# Autodesk Inventor assembly: ModuleFold
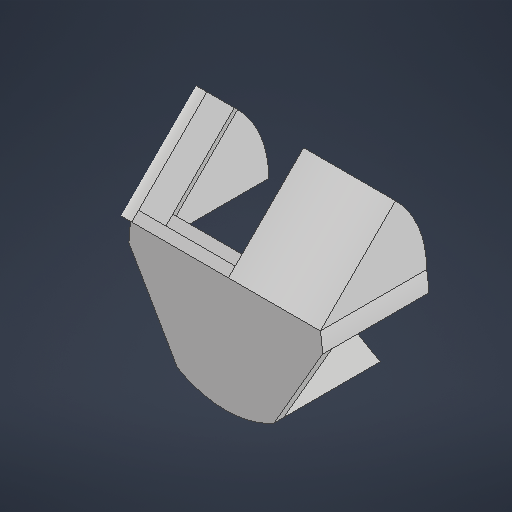
[picture p0: Inventor's stored thumbnail of the model, 512x512]
Saved by Autodesk Inventor 2026.2 (Build 302298000, 298)
## iProperties
Created: 2026-06-17
Part Number: ModuleFold
Document SubType Name: Assembly
Designer: Jakub Schmidt
Author: Jakub Schmidt
## Documents named in this file (3)
- C:\Users\Jakub Schmidt\Desktop\100M_SA\SG\10mm (Recent)\2x2mm(Recent)\2DFolded\BeetleDarhani\ModuleFold.iam
- C:\Users\Jakub Schmidt\Desktop\100M_SA\SG\10mm (Recent)\2x2mm(Recent)\2DFolded\BeetleDarhani\BodyFoldedSide1.ipt
- C:\Users\Jakub Schmidt\Desktop\100M_SA\SG\10mm (Recent)\2x2mm(Recent)\2DFolded\BeetleDarhani\BodyFoldedSide2.ipt
## Components (2 placed, 2 different names)
1. BodyFoldedSide1:1 — Mate:1, Mate:2, Mate:3
2. BodyFoldedSide2:1 — Mate:1, Mate:2, Mate:3
## Relationships (3: Mate 3)
- Mate:1: BodyFoldedSide1:1 ↔ BodyFoldedSide2:1
- Mate:2: BodyFoldedSide1:1 ↔ BodyFoldedSide2:1
- Mate:3: BodyFoldedSide1:1 ↔ BodyFoldedSide2:1
